# Autodesk Inventor assembly: prototype_5_batteryWithSlider
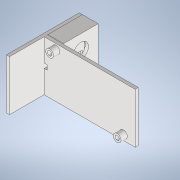
[picture p0: Inventor's stored thumbnail of the model, 180x180]
Saved by Autodesk Inventor 2022 (Build 260153000, 153)
## iProperties
Created: 2022-06-08
Part Number: prototype_5_batteryWithSlider
Document SubType Name: Assembly
Designer: tecware
Author: tecware
## Documents named in this file (4)
- C:\Users\tecware\Documents\git\calibrationKit\calibrationKit_v2\wand\prototype\prototype_5_batteryWithSlider.iam
- C:\Users\tecware\Documents\git\calibrationKit\calibrationKit_v2\wand\prototype\prototype_5_batteryPart.ipt
- C:\Users\tecware\Documents\git\calibrationKit\calibrationKit_v2\wand\prototype\prototype_5_sliderPart.ipt
- C:\Users\tecware\Documents\git\calibrationKit\calibrationKit_v2\wand\prototype\prototype_5_testPart1.ipt
## Components (3 placed, 3 different names)
1. prototype_5_batteryPart:1 — Flush:1, Mate:1, Mate:2, Mate:3, Flush:4, Flush:5
2. prototype_5_sliderPart:1 — Flush:1, Mate:1, Mate:2
3. prototype_5_testPart1:1 — Mate:3, Flush:4, Flush:5
## Relationships (6: Flush 3, Mate 3)
- Flush:1: prototype_5_batteryPart:1 ↔ prototype_5_sliderPart:1
- Mate:1 (0.2 mm): prototype_5_batteryPart:1 ↔ prototype_5_sliderPart:1
- Mate:2 (0.2 mm): prototype_5_batteryPart:1 ↔ prototype_5_sliderPart:1
- Mate:3: prototype_5_batteryPart:1 ↔ prototype_5_testPart1:1
- Flush:4: prototype_5_batteryPart:1 ↔ prototype_5_testPart1:1
- Flush:5: prototype_5_batteryPart:1 ↔ prototype_5_testPart1:1
